# Autodesk Inventor assembly: Butterfly Drive Module_MIR1
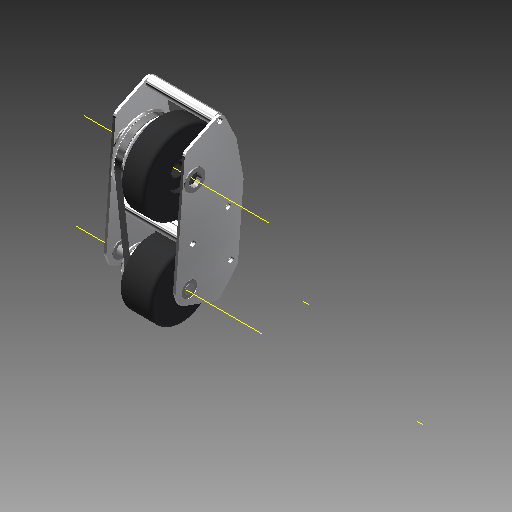
[picture p0: Inventor's stored thumbnail of the model, 512x512]
Saved by Autodesk Inventor 2019.4 (Build 234330000, 330)
## iProperties
Created: 2019-10-18
Part Number: Butterfly Drive Module_MIR1
Document SubType Name: Assembly
Designer: admin
Author: admin
## Documents named in this file (11)
- C:\Users\admin\Desktop\FRC 2020 Engineering\GitHub\7738-CAD-prep\Butterfly drive\Butterfly Drive Module_MIR1.iam
- C:\Users\admin\Desktop\FRC 2020 Engineering\GitHub\7738-CAD-prep\Butterfly drive\Connector_MIR.ipt
- C:\Users\admin\Desktop\FRC 2020 Engineering\GitHub\7738-CAD-prep\Butterfly drive\100mm Mecanum StandIn_MIR1.ipt
- C:\Users\admin\Desktop\FRC 2020 Engineering\GitHub\7738-CAD-prep\Butterfly drive\100mm Traction Wheel StandIn_MIR1.ipt
- C:\Users\admin\Desktop\FRC 2020 Engineering\GitHub\7738-CAD-prep\Butterfly drive\Butterfly Drive Module\Design Accelerator\Synchronous Belts Transmission3_MIR1.iam
- C:\Users\admin\Desktop\FRC 2020 Engineering\GitHub\7738-CAD-prep\Butterfly drive\Module Plate 1_MIR1.ipt
- C:\Users\admin\Desktop\FRC 2020 Engineering\GitHub\7738-CAD-prep\Butterfly drive\F6004_MIR.ipt
- C:\Users\admin\Desktop\FRC 2020 Engineering\GitHub\7738-CAD-prep\Butterfly drive\F6802_MIR.ipt
- C:\Users\admin\Desktop\FRC 2020 Engineering\GitHub\7738-CAD-prep\Butterfly drive\Butterfly Drive Module\Design Accelerator\Shaft1_MIR.iam
- C:\Users\admin\Desktop\FRC 2020 Engineering\GitHub\7738-CAD-prep\Butterfly drive\M6GBTeye_MIR.ipt
- C:\Users\admin\Desktop\FRC 2020 Engineering\GitHub\7738-CAD-prep\Butterfly drive\Butterfly Drive Module\Design Accelerator\Shaft3_MIR.iam
## Components (17 placed, 10 different names)
1. Connector_MIR:1 — Mate:66, Mate:64, Mate:34, Mate:49
2. 100mm Mecanum StandIn_MIR1:1 — Flush:1, Mate:5, Mate:37, Angle:1, Mate:42
3. 100mm Traction Wheel StandIn_MIR1:1 — Flush:1, Mate:4, Mate:6
4. Synchronous Belts Transmission3_MIR1:1 [sub-assembly] — Mate:5, Mate:37, Mate:6, Mate:41, Angle:2, Mate:40
5. Module Plate 1_MIR1:1 — Mate:42, Mate:41, Flush:3, Flush:2, Mate:33, Mate:66, Mate:64, Mate:58, Mate:57, Mate:55, Mate:52, Mate:39, Mate:44, Mate:43, Mate:46, Mate:45, Mate:67, Mate:65
6. Module Plate 1_MIR1:2 — Angle:2, Flush:3, Flush:2, Mate:33, Mate:60, Mate:59, Mate:54, Mate:53, Mate:50
7. F6004_MIR:1 — Mate:60, Mate:59
8. F6004_MIR:2 — Mate:58, Mate:57
9. F6802_MIR:1 — Mate:54, Mate:53
10. F6802_MIR:2 — Mate:55, Mate:52, Flush:4, Mate:61
11. Connector_MIR:2 — Mate:44, Mate:43
12. Shaft1_MIR:1 [sub-assembly] — Flush:4, Mate:61
13. Connector_MIR:3 — Mate:46, Mate:45
14. M6GBTeye_MIR:1 — Mate:50, Mate:49, Mate:47, Mate:62, Mate:51
15. M6GBTeye_MIR:2 — Mate:47, Mate:48, Mate:63
16. Connector_MIR:4 — Mate:67, Mate:65, Mate:48
17. Shaft3_MIR:1 [sub-assembly] — Mate:63, Mate:62
## Relationships (40: Mate 34, Flush 4, Angle 2)
- Flush:1 (10.5 mm): 100mm Mecanum StandIn_MIR1:1 ↔ 100mm Traction Wheel StandIn_MIR1:1
- Mate:4: 100mm Traction Wheel StandIn_MIR1:1
- Mate:5: 100mm Mecanum StandIn_MIR1:1 ↔ Synchronous Belts Transmission3_MIR1:1
- Mate:37 (2 mm): 100mm Mecanum StandIn_MIR1:1 ↔ Synchronous Belts Transmission3_MIR1:1
- Angle:1 (-90 deg): 100mm Mecanum StandIn_MIR1:1
- Mate:6: 100mm Traction Wheel StandIn_MIR1:1 ↔ Synchronous Belts Transmission3_MIR1:1
- Mate:42 (3.5 mm): 100mm Mecanum StandIn_MIR1:1 ↔ Module Plate 1_MIR1:1
- Mate:41: Synchronous Belts Transmission3_MIR1:1 ↔ Module Plate 1_MIR1:1
- Angle:2 (180 deg): Synchronous Belts Transmission3_MIR1:1 ↔ Module Plate 1_MIR1:2
- Flush:3: Module Plate 1_MIR1:1 ↔ Module Plate 1_MIR1:2
- Flush:2: Module Plate 1_MIR1:1 ↔ Module Plate 1_MIR1:2
- Mate:33 (105 mm): Module Plate 1_MIR1:1 ↔ Module Plate 1_MIR1:2
- Mate:66 (0.3 mm): Connector_MIR:1 ↔ Module Plate 1_MIR1:1
- Mate:64: Connector_MIR:1 ↔ Module Plate 1_MIR1:1
- Mate:34: Connector_MIR:1
- Mate:60 (0.2 mm): Module Plate 1_MIR1:2 ↔ F6004_MIR:1
- Mate:59: Module Plate 1_MIR1:2 ↔ F6004_MIR:1
- Mate:58 (0.2 mm): Module Plate 1_MIR1:1 ↔ F6004_MIR:2
- Mate:57: Module Plate 1_MIR1:1 ↔ F6004_MIR:2
- Mate:54 (0.2 mm): Module Plate 1_MIR1:2 ↔ F6802_MIR:1
- Mate:53: Module Plate 1_MIR1:2 ↔ F6802_MIR:1
- Mate:55 (0.2 mm): Module Plate 1_MIR1:1 ↔ F6802_MIR:2
- Mate:52: Module Plate 1_MIR1:1 ↔ F6802_MIR:2
- Mate:40: Synchronous Belts Transmission3_MIR1:1
- Mate:39: Module Plate 1_MIR1:1
- Mate:44: Module Plate 1_MIR1:1 ↔ Connector_MIR:2
- Mate:43: Module Plate 1_MIR1:1 ↔ Connector_MIR:2
- Flush:4 (-0.2 mm): F6802_MIR:2 ↔ Shaft1_MIR:1
- Mate:61: F6802_MIR:2 ↔ Shaft1_MIR:1
- Mate:46: Module Plate 1_MIR1:1 ↔ Connector_MIR:3
- Mate:45: Module Plate 1_MIR1:1 ↔ Connector_MIR:3
- Mate:50 (58.5 mm): Module Plate 1_MIR1:2 ↔ M6GBTeye_MIR:1
- Mate:49: Connector_MIR:1 ↔ M6GBTeye_MIR:1
- Mate:47: M6GBTeye_MIR:1 ↔ M6GBTeye_MIR:2
- Mate:67 (0.3 mm): Module Plate 1_MIR1:1 ↔ Connector_MIR:4
- Mate:65: Module Plate 1_MIR1:1 ↔ Connector_MIR:4
- Mate:48: M6GBTeye_MIR:2 ↔ Connector_MIR:4
- Mate:63 (3 mm): M6GBTeye_MIR:2 ↔ Shaft3_MIR:1
- Mate:62: M6GBTeye_MIR:1 ↔ Shaft3_MIR:1
- Mate:51: M6GBTeye_MIR:1
